# Autodesk Inventor assembly: Button Panel Assembly
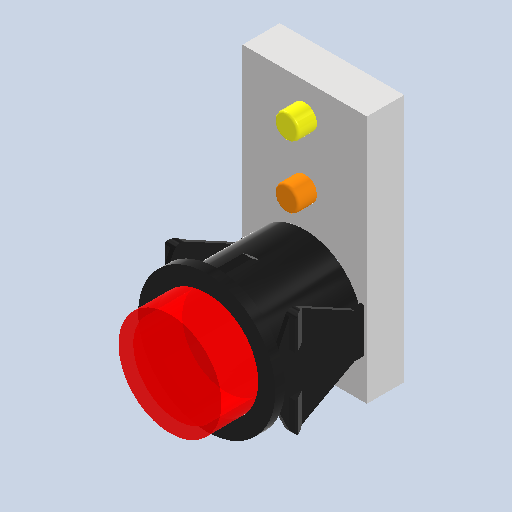
[picture p0: Inventor's stored thumbnail of the model, 512x512]
Saved by Autodesk Inventor 2022 (Build 260153000, 153)
## iProperties
Created: 2023-05-17
Part Number: Button Panel Assembly
Document SubType Name: Assembly
Designer: brenden_deutschman
Description: Powerbutton, On Light, and Hot Light
Author: brenden_deutschman
Title: Button Panel Subassembly
## Documents named in this file (5)
- G:\Documents\Inventor HW\Hexagonal_Hive\Button Panel Assembly.iam
- G:\Documents\Inventor HW\Hexagonal_Hive\PS18-16 push lached button\Button Panel.ipt
- G:\Documents\Inventor HW\Hexagonal_Hive\PS18-16 push lached button\PS18-16 assy.iam
- G:\Documents\Inventor HW\Hexagonal_Hive\PS18-16 push lached button\Mini Lights.ipt
- G:\Documents\Inventor HW\Hexagonal_Hive\PS18-16 push lached button\Mini Lights Yellow.ipt
## Components (4 placed, 4 different names)
1. Button Panel:1 — Rotational:1, Rotational:2, Cylindrical:1
2. PS18-16 assy:1 [sub-assembly] — Cylindrical:1
3. Mini Lights:1 — Rotational:2
4. Mini Lights Yellow:1 — Rotational:1
## Relationships (3: RevoluteJoint 2, CylindricalJoint 1)
- Rotational:1 [RevoluteJoint] (1.27 mm): Button Panel:1 ↔ Mini Lights Yellow:1
- Rotational:2 [RevoluteJoint] (1.27 mm): Button Panel:1 ↔ Mini Lights:1
- Cylindrical:1: Button Panel:1 ↔ PS18-16 assy:1
